# Autodesk Inventor assembly: PeepAsmV4
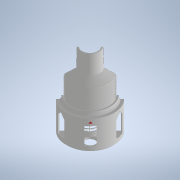
[picture p0: Inventor's stored thumbnail of the model, 180x180]
Saved by Autodesk Inventor 2020 (Build 240168000, 168)
## iProperties
Created: 2020-05-16
Part Number: PeepAsmV4
Document SubType Name: Assembly
Designer: Theo Cominotto
Author: Theo Cominotto
## Documents named in this file (8)
- C:\Users\Theo Cominotto\Dropbox\Beademingstoestel VUB\Beademingstoestel VUB-PEEP VALVE\Peep Custom\PeepAsmV4.iam
- C:\Users\Theo Cominotto\Dropbox\Beademingstoestel VUB\Beademingstoestel VUB-PEEP VALVE\Peep Custom\PeepBaseV4.ipt
- C:\Users\Theo Cominotto\Dropbox\Beademingstoestel VUB\Beademingstoestel VUB-PEEP VALVE\Peep Custom\PeepCoverV4.ipt
- C:\Users\Theo Cominotto\Dropbox\Beademingstoestel VUB\Beademingstoestel VUB-PEEP VALVE\Peep Custom\Seal_M_TPU.ipt
- C:\Users\Theo Cominotto\Dropbox\Beademingstoestel VUB\Beademingstoestel VUB-PEEP VALVE\Peep Custom\Seal_M.ipt
- C:\Users\Theo Cominotto\Dropbox\Beademingstoestel VUB\Beademingstoestel VUB-PEEP VALVE\Peep Custom\M3Rod.ipt
- C:\Users\Theo Cominotto\Dropbox\Beademingstoestel VUB\Beademingstoestel VUB-PEEP VALVE\Peep Custom\Spring.ipt
- C:\Users\Theo Cominotto\Documents\Inventor\Content Center Files\R2020\en-US\DIN 934\DIN 934 - M3 x 0,5.ipt
## Components (8 placed, 7 different names)
1. PeepBaseV4:1 — Mate:1, Mate:2, Mate:3, Mate:4, Mate:7, Mate:8
2. PeepCoverV4:1 — Mate:2, Mate:9, Mate:10
3. Seal_M_TPU:1 — Mate:3, Mate:5, Mate:12, Mate:14
4. Seal_M:1 — Mate:4, Mate:5
5. M3Rod:1 — Mate:7, Mate:8, Mate:13
6. Spring:1 — Mate:9, Mate:10, Mate:11, Mate:15
7. DIN 934 - replaced by DIN EN 24032/28673/28674 M3:1 — Mate:13, Mate:14
8. DIN 934 - replaced by DIN EN 24032/28673/28674 M3:2 — Mate:11, Mate:12
## Relationships (17: Mate 15, Angle 2)
- Mate:1: PeepBaseV4:1
- Mate:2: PeepBaseV4:1 ↔ PeepCoverV4:1
- Mate:3: PeepBaseV4:1 ↔ Seal_M_TPU:1
- Mate:4: PeepBaseV4:1 ↔ Seal_M:1
- Mate:5: Seal_M_TPU:1 ↔ Seal_M:1
- Mate:6
- Angle:1 (45 deg)
- Mate:7: PeepBaseV4:1 ↔ M3Rod:1
- Mate:8: PeepBaseV4:1 ↔ M3Rod:1
- Mate:9: PeepCoverV4:1 ↔ Spring:1
- Mate:10: PeepCoverV4:1 ↔ Spring:1
- Mate:11: Spring:1 ↔ DIN 934 - replaced by DIN EN 24032/28673/28674 M3:2
- Mate:12: Seal_M_TPU:1 ↔ DIN 934 - replaced by DIN EN 24032/28673/28674 M3:2
- Mate:13: M3Rod:1 ↔ DIN 934 - replaced by DIN EN 24032/28673/28674 M3:1
- Mate:14: Seal_M_TPU:1 ↔ DIN 934 - replaced by DIN EN 24032/28673/28674 M3:1
- Mate:15: Spring:1
- Angle:2 (45 deg)
